# Autodesk Inventor assembly: CAM11
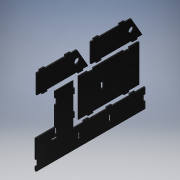
[picture p0: Inventor's stored thumbnail of the model, 180x180]
Saved by Autodesk Inventor 2017 (Build 210142000, 142)
## iProperties
Created: 2019-06-07
Part Number: CAM11
Document SubType Name: Assembly
Designer: Dell
Author: Dell
## Documents named in this file (4)
- C:\Users\Dell\Documents\GitHub\tr2\Body 2.0\CAM11.iam
- C:\Users\Dell\Documents\GitHub\tr2\Body 2.0\BA10.ipt
- C:\Users\Dell\Documents\GitHub\tr2\Body 2.0\BA17b.ipt
- C:\Users\Dell\Documents\GitHub\tr2\Body 2.0\BA23.ipt
## Components (4 placed, 3 different names)
1. BA10:1 — Flush:2, Angle:1, Flush:3, Flush:4, Angle:2, Angle:3
2. BA17b:1 — Flush:2, Angle:1
3. BA23:1 — Flush:4, Angle:2
4. BA23:2 — Flush:3, Angle:3
## Relationships (6: Flush 3, Angle 3)
- Flush:2: BA10:1 ↔ BA17b:1
- Angle:1 (0 deg): BA10:1 ↔ BA17b:1
- Flush:3: BA10:1 ↔ BA23:2
- Flush:4: BA10:1 ↔ BA23:1
- Angle:2 (0 deg): BA10:1 ↔ BA23:1
- Angle:3 (0 deg): BA10:1 ↔ BA23:2
## Named parameters: Fit_Tolerance = 1.27 mm
